# Autodesk Inventor assembly: Grippera
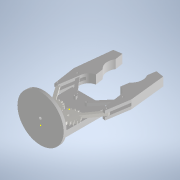
[picture p0: Inventor's stored thumbnail of the model, 180x180]
Saved by Autodesk Inventor 2022 (Build 260153000, 153)
## iProperties
Created: 2022-01-15
Part Number: Grippera
Document SubType Name: Assembly
Designer: nguye
Author: nguye
## Documents named in this file (5)
- G:\My Drive\Study\Semester 5\Roboty Uslugowe\Project\Model\Grippera.iam
- G:\My Drive\Study\Semester 5\Roboty Uslugowe\Project\Model\Gear.ipt
- G:\My Drive\Study\Semester 5\Roboty Uslugowe\Project\Model\gripper.ipt
- G:\My Drive\Study\Semester 5\Roboty Uslugowe\Project\Model\gripper1.ipt
- G:\My Drive\Study\Semester 5\Roboty Uslugowe\Project\Model\gripper3.ipt
## Components (7 placed, 4 different names)
1. gripper:1 — Mate:5, Mate:6, Mate:7, Mate:8, Mate:14, Mate:15, Mate:17, Mate:18
2. gripper1:1 — Mate:5, Mate:6, Mate:12, Mate:13
3. gripper3:1 — Mate:11, Mate:16
4. gripper1:2 — Mate:7, Mate:8, Mate:11
5. gripper3:2 — Mate:12, Mate:13, Mate:19
6. Spur Gear1:1 — Mate:14, Mate:15, Mate:16
7. Spur Gear1:2 — Mate:17, Mate:18, Mate:19
## Relationships (13: Mate 13)
- Mate:5: gripper:1 ↔ gripper1:1
- Mate:6: gripper:1 ↔ gripper1:1
- Mate:7: gripper:1 ↔ gripper1:2
- Mate:8: gripper:1 ↔ gripper1:2
- Mate:11: gripper3:1 ↔ gripper1:2
- Mate:12: gripper1:1 ↔ gripper3:2
- Mate:13: gripper1:1 ↔ gripper3:2
- Mate:14: gripper:1 ↔ Spur Gear1:1
- Mate:15: gripper:1 ↔ Spur Gear1:1
- Mate:16: gripper3:1 ↔ Spur Gear1:1
- Mate:17: gripper:1 ↔ Spur Gear1:2
- Mate:18: gripper:1 ↔ Spur Gear1:2
- Mate:19: gripper3:2 ↔ Spur Gear1:2
